# Autodesk Inventor assembly: Completo
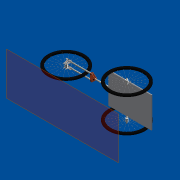
[picture p0: Inventor's stored thumbnail of the model, 180x180]
Saved by Autodesk Inventor 2016 (Build 200138000, 138)
## iProperties
Created: 2017-05-13
Part Number: Completo
Document SubType Name: Assembly
Designer: Gian
Author: Gian
## Documents named in this file (5)
- C:\Users\Gian\Desktop\Pedalazo\002_Diseño\Version_001\Completo.iam
- C:\Users\Gian\Desktop\Pedalazo\002_Diseño\Version_001\Rueda.ipt
- C:\Users\Gian\Desktop\Pedalazo\002_Diseño\Version_001\Tubo_conexion.ipt
- C:\Users\Gian\Desktop\Pedalazo\002_Diseño\Version_001\tren.iam
- C:\Users\Gian\Desktop\Pedalazo\002_Diseño\Version_001\Carro.iam
## Components (4 placed, 4 different names)
1. Rueda:1
2. Tubo_conexion:2 — Cylindrical:1
3. tren:1 [sub-assembly] — Flush:5, Cylindrical:1
4. Carro:1 [sub-assembly]
## Relationships (2: Flush 1, CylindricalJoint 1)
- Flush:5: tren:1
- Cylindrical:1: Tubo_conexion:2 ↔ tren:1
